# Autodesk Inventor assembly: assemblage_base_amovible
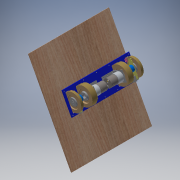
[picture p0: Inventor's stored thumbnail of the model, 180x180]
Saved by Autodesk Inventor 2017 (Build 210142000, 142)
## iProperties
Created: 2017-04-12
Part Number: assemblage_base_amovible
Document SubType Name: Assembly
Designer: franc
Author: franc
## Documents named in this file (13)
- C:\Users\franc\Desktop\EsialRobotik\Mecanique\base roulante\assemblage_base_amovible.iam
- C:\Users\franc\Desktop\EsialRobotik\Mecanique\base roulante\base_roulante.ipt
- C:\Users\franc\Desktop\EsialRobotik\Mecanique\base roulante\support_moteur.ipt
- C:\Users\franc\Desktop\EsialRobotik\Mecanique\base roulante\37d-gearmotor-19-30.ipt
- C:\Users\franc\Desktop\EsialRobotik\Mecanique\base roulante\moyeu_serrage_conique.ipt
- C:\Users\franc\Desktop\EsialRobotik\Mecanique\base roulante\Colson_Wheel_3in_x_7_8in.ipt
- C:\Users\franc\Desktop\EsialRobotik\Mecanique\base roulante\palier_roulement_bras.ipt
- C:\Users\franc\Desktop\EsialRobotik\Mecanique\base roulante\bras_amortisseur.ipt
- C:\Users\franc\Desktop\EsialRobotik\Mecanique\base roulante\Codeur.ipt
- C:\Users\franc\Desktop\EsialRobotik\Mecanique\base roulante\T40_hub_40mm_1screw.ipt
- C:\Users\franc\Desktop\EsialRobotik\Mecanique\base roulante\T40_Wheel_2_875in_x_0_5in.ipt
- C:\Users\franc\Desktop\EsialRobotik\Mecanique\base roulante\sol.ipt
- C:\Users\franc\Desktop\EsialRobotik\Mecanique\base roulante\crochet.ipt
## Components (22 placed, 12 different names)
1. base_roulante:1 — Mate:1, Mate:2, Mate:3, Mate:4, Mate:5, Mate:6, Mate:19, Mate:20, Mate:21, Mate:22, Mate:23, Mate:24, Angle:1, Flush:3, Flush:4, Mate:46, Mate:48
2. support_moteur:1 — Mate:1, Mate:2, Mate:3, Mate:7, Mate:8, Mate:9
3. support_moteur:2 — Mate:4, Mate:5, Mate:6, Mate:10, Mate:11, Mate:12
4. 37d-gearmotor-19-30:1 — Mate:10, Mate:11, Mate:12, Mate:13, Mate:14
5. 37d-gearmotor-19-30:2 — Mate:7, Mate:8, Mate:9, Mate:15, Mate:16
6. moyeu_serrage_conique:1 — Mate:13, Mate:14, Mate:18, Flush:2
7. moyeu_serrage_conique:2 — Mate:15, Mate:16, Mate:17, Flush:1
8. Colson_Wheel_3in_x_7_8in:1 — Mate:17, Flush:1, Mate:43, Tangent:1
9. Colson_Wheel_3in_x_7_8in:2 — Mate:18, Flush:2, Mate:44
10. palier_roulement_bras:1 — Mate:19, Mate:20, Mate:21, Mate:28, Mate:29
11. palier_roulement_bras:2 — Mate:22, Mate:23, Mate:24, Mate:30, Mate:31
12. bras_amortisseur:1 — Mate:25, Mate:26, Mate:27, Mate:28, Mate:29, Mate:36, Mate:47, Flush:7
13. bras_amortisseur:2 — Mate:30, Mate:31, Mate:32, Mate:33, Mate:34, Mate:38, Flush:5, Mate:45
14. Codeur:1 — Mate:25, Mate:26, Mate:27, Mate:35
15. Codeur:2 — Mate:32, Mate:33, Mate:34, Mate:37
16. T40_hub_40mm_1screw:1 — Mate:35, Mate:36, Mate:39, Mate:40
17. T40_hub_40mm_1screw:2 — Mate:37, Mate:38, Mate:41, Mate:42
18. T40_Wheel_2_875in_x_0_5in:1 — Mate:39, Mate:40
19. T40_Wheel_2_875in_x_0_5in:2 — Mate:41, Mate:42
20. sol:1 — Mate:43, Mate:44, Angle:1, Flush:3, Tangent:1, Flush:4
21. crochet:1 — Flush:5, Mate:45, Mate:46
22. crochet:2 — Mate:47, Mate:48, Flush:7
## Relationships (56: Mate 48, Flush 6, Angle 1, Tangent 1)
- Mate:1: base_roulante:1 ↔ support_moteur:1
- Mate:2: base_roulante:1 ↔ support_moteur:1
- Mate:3: base_roulante:1 ↔ support_moteur:1
- Mate:4: base_roulante:1 ↔ support_moteur:2
- Mate:5: base_roulante:1 ↔ support_moteur:2
- Mate:6: base_roulante:1 ↔ support_moteur:2
- Mate:7: support_moteur:1 ↔ 37d-gearmotor-19-30:2
- Mate:8: support_moteur:1 ↔ 37d-gearmotor-19-30:2
- Mate:9: support_moteur:1 ↔ 37d-gearmotor-19-30:2
- Mate:10: support_moteur:2 ↔ 37d-gearmotor-19-30:1
- Mate:11: support_moteur:2 ↔ 37d-gearmotor-19-30:1
- Mate:12: support_moteur:2 ↔ 37d-gearmotor-19-30:1
- Mate:13: 37d-gearmotor-19-30:1 ↔ moyeu_serrage_conique:1
- Mate:14: 37d-gearmotor-19-30:1 ↔ moyeu_serrage_conique:1
- Mate:15: 37d-gearmotor-19-30:2 ↔ moyeu_serrage_conique:2
- Mate:16: 37d-gearmotor-19-30:2 ↔ moyeu_serrage_conique:2
- Mate:17: moyeu_serrage_conique:2 ↔ Colson_Wheel_3in_x_7_8in:1
- Flush:1: moyeu_serrage_conique:2 ↔ Colson_Wheel_3in_x_7_8in:1
- Mate:18: moyeu_serrage_conique:1 ↔ Colson_Wheel_3in_x_7_8in:2
- Flush:2: moyeu_serrage_conique:1 ↔ Colson_Wheel_3in_x_7_8in:2
- Mate:19: base_roulante:1 ↔ palier_roulement_bras:1
- Mate:20: base_roulante:1 ↔ palier_roulement_bras:1
- Mate:21: base_roulante:1 ↔ palier_roulement_bras:1
- Mate:22: base_roulante:1 ↔ palier_roulement_bras:2
- Mate:23: base_roulante:1 ↔ palier_roulement_bras:2
- Mate:24: base_roulante:1 ↔ palier_roulement_bras:2
- Mate:25: bras_amortisseur:1 ↔ Codeur:1
- Mate:26: bras_amortisseur:1 ↔ Codeur:1
- Mate:27: bras_amortisseur:1 ↔ Codeur:1
- Mate:28: palier_roulement_bras:1 ↔ bras_amortisseur:1
- Mate:29: palier_roulement_bras:1 ↔ bras_amortisseur:1
- Mate:30: palier_roulement_bras:2 ↔ bras_amortisseur:2
- Mate:31: palier_roulement_bras:2 ↔ bras_amortisseur:2
- Mate:32: bras_amortisseur:2 ↔ Codeur:2
- Mate:33: bras_amortisseur:2 ↔ Codeur:2
- Mate:34: bras_amortisseur:2 ↔ Codeur:2
- Mate:35: Codeur:1 ↔ T40_hub_40mm_1screw:1
- Mate:36 (1 mm): bras_amortisseur:1 ↔ T40_hub_40mm_1screw:1
- Mate:37: Codeur:2 ↔ T40_hub_40mm_1screw:2
- Mate:38 (1 mm): bras_amortisseur:2 ↔ T40_hub_40mm_1screw:2
- Mate:39: T40_hub_40mm_1screw:1 ↔ T40_Wheel_2_875in_x_0_5in:1
- Mate:40: T40_hub_40mm_1screw:1 ↔ T40_Wheel_2_875in_x_0_5in:1
- Mate:41: T40_hub_40mm_1screw:2 ↔ T40_Wheel_2_875in_x_0_5in:2
- Mate:42: T40_hub_40mm_1screw:2 ↔ T40_Wheel_2_875in_x_0_5in:2
- Mate:43: Colson_Wheel_3in_x_7_8in:1 ↔ sol:1
- Mate:44: Colson_Wheel_3in_x_7_8in:2 ↔ sol:1
- Angle:1 (0 deg): base_roulante:1 ↔ sol:1
- Flush:3 (150 mm): base_roulante:1 ↔ sol:1
- Tangent:1: Colson_Wheel_3in_x_7_8in:1 ↔ sol:1
- Flush:4: base_roulante:1 ↔ sol:1
- Flush:5: bras_amortisseur:2 ↔ crochet:1
- Mate:45: bras_amortisseur:2 ↔ crochet:1
- Mate:46: base_roulante:1 ↔ crochet:1
- Mate:47: bras_amortisseur:1 ↔ crochet:2
- Mate:48: base_roulante:1 ↔ crochet:2
- Flush:7: bras_amortisseur:1 ↔ crochet:2
